# Autodesk Inventor assembly: 101_CompCellScopeAssembly
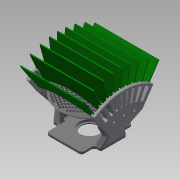
[picture p0: Inventor's stored thumbnail of the model, 180x180]
Saved by Autodesk Inventor 2015 (Build 190159000, 159)
## iProperties
Created: 2015-01-06
Part Number: 101_CompCellScopeAssembly
Document SubType Name: Assembly
Designer: Zack
Author: Zack
## Documents named in this file (6)
- C:\Users\Zack\Dropbox\LED_Array_CellScope\OpenSource\CAD Designs\Inventor\For Submission\101_CompCellScopeAssembly.iam
- C:\Users\Zack\Dropbox\LED_Array_CellScope\OpenSource\CAD Designs\Inventor\For Submission\102_CompCellScopeDome.ipt
- C:\Users\Zack\Dropbox\LED_Array_CellScope\OpenSource\CAD Designs\Inventor\For Submission\103_CompCellScopeStage.ipt
- C:\Users\Zack\Dropbox\LED_Array_CellScope\OpenSource\CAD Designs\Inventor\For Submission\104_CompCellScopeBoardHolder.ipt
- C:\Users\Zack\Dropbox\LED_Array_CellScope\OpenSource\CAD Designs\Inventor\For Submission\901_CompCellScopeBoard_FORPICS.ipt
- C:\Users\Zack\Dropbox\LED_Array_CellScope\OpenSource\CAD Designs\Inventor\For Submission\902_CompCellScopeLED_FORPICS.ipt
## Components (14 placed, 5 different names)
1. 102_CompCellScopeDome:1 — Mate:1, Angle:1, Angle:2, Mate:2, Mate:3, Mate:4, Mate:38, Mate:39
2. 103_CompCellScopeStage:1 — Mate:2, Mate:3, Mate:4, Mate:6
3. 104_CompCellScopeBoardHolder:1 — Mate:6, Mate:7, Angle:3, Mate:27, Mate:28, Mate:29, Mate:30, Mate:31, Mate:32, Mate:34, Mate:35
4. 104_CompCellScopeBoardHolder:2 — Mate:8, Mate:9, Flush:1, Mate:10, Mate:11, Mate:12, Mate:13, Mate:14, Mate:15, Mate:16, Mate:17, Mate:18, Mate:19, Mate:20, Mate:21, Mate:22, Mate:23, Mate:24, Mate:25, Mate:26, Mate:33, Mate:36, Mate:37
5. 901_CompCellScopeBoard_FORPICS:1 — Mate:10, Mate:11, Mate:12
6. 901_CompCellScopeBoard_FORPICS:2 — Mate:17, Mate:18, Mate:19
7. 901_CompCellScopeBoard_FORPICS:3 — Mate:20, Mate:21, Mate:22
8. 901_CompCellScopeBoard_FORPICS:4 — Mate:13, Mate:14, Mate:15, Mate:16
9. 901_CompCellScopeBoard_FORPICS:5 — Mate:23, Mate:24, Mate:25
10. 901_CompCellScopeBoard_FORPICS:6 — Mate:31, Mate:32, Mate:36
11. 901_CompCellScopeBoard_FORPICS:7 — Mate:29, Mate:30, Mate:37
12. 901_CompCellScopeBoard_FORPICS:8 — Mate:26, Mate:27, Mate:28
13. 901_CompCellScopeBoard_FORPICS:9 — Mate:33, Mate:34, Mate:35
14. 902_CompCellScopeLED_FORPICS:1 — Mate:38, Mate:39
## Relationships (42: Mate 38, Angle 3, Flush 1)
- Mate:1: 102_CompCellScopeDome:1
- Angle:1 (0 deg): 102_CompCellScopeDome:1
- Angle:2 (0 deg): 102_CompCellScopeDome:1
- Mate:2: 102_CompCellScopeDome:1 ↔ 103_CompCellScopeStage:1
- Mate:3: 102_CompCellScopeDome:1 ↔ 103_CompCellScopeStage:1
- Mate:4: 102_CompCellScopeDome:1 ↔ 103_CompCellScopeStage:1
- Mate:6: 103_CompCellScopeStage:1 ↔ 104_CompCellScopeBoardHolder:1
- Mate:7: 104_CompCellScopeBoardHolder:1
- Angle:3 (0 deg): 104_CompCellScopeBoardHolder:1
- Mate:8: 104_CompCellScopeBoardHolder:2
- Mate:9: 104_CompCellScopeBoardHolder:2
- Flush:1: 104_CompCellScopeBoardHolder:2
- Mate:10: 104_CompCellScopeBoardHolder:2 ↔ 901_CompCellScopeBoard_FORPICS:1
- Mate:11: 104_CompCellScopeBoardHolder:2 ↔ 901_CompCellScopeBoard_FORPICS:1
- Mate:12: 104_CompCellScopeBoardHolder:2 ↔ 901_CompCellScopeBoard_FORPICS:1
- Mate:13: 104_CompCellScopeBoardHolder:2 ↔ 901_CompCellScopeBoard_FORPICS:4
- Mate:14: 104_CompCellScopeBoardHolder:2 ↔ 901_CompCellScopeBoard_FORPICS:4
- Mate:15: 104_CompCellScopeBoardHolder:2 ↔ 901_CompCellScopeBoard_FORPICS:4
- Mate:16: 104_CompCellScopeBoardHolder:2 ↔ 901_CompCellScopeBoard_FORPICS:4
- Mate:17: 104_CompCellScopeBoardHolder:2 ↔ 901_CompCellScopeBoard_FORPICS:2
- Mate:18: 104_CompCellScopeBoardHolder:2 ↔ 901_CompCellScopeBoard_FORPICS:2
- Mate:19: 104_CompCellScopeBoardHolder:2 ↔ 901_CompCellScopeBoard_FORPICS:2
- Mate:20: 104_CompCellScopeBoardHolder:2 ↔ 901_CompCellScopeBoard_FORPICS:3
- Mate:21: 104_CompCellScopeBoardHolder:2 ↔ 901_CompCellScopeBoard_FORPICS:3
- Mate:22: 104_CompCellScopeBoardHolder:2 ↔ 901_CompCellScopeBoard_FORPICS:3
- Mate:23: 104_CompCellScopeBoardHolder:2 ↔ 901_CompCellScopeBoard_FORPICS:5
- Mate:24: 104_CompCellScopeBoardHolder:2 ↔ 901_CompCellScopeBoard_FORPICS:5
- Mate:25: 104_CompCellScopeBoardHolder:2 ↔ 901_CompCellScopeBoard_FORPICS:5
- Mate:26: 104_CompCellScopeBoardHolder:2 ↔ 901_CompCellScopeBoard_FORPICS:8
- Mate:27: 104_CompCellScopeBoardHolder:1 ↔ 901_CompCellScopeBoard_FORPICS:8
- Mate:28: 104_CompCellScopeBoardHolder:1 ↔ 901_CompCellScopeBoard_FORPICS:8
- Mate:29: 104_CompCellScopeBoardHolder:1 ↔ 901_CompCellScopeBoard_FORPICS:7
- Mate:30: 104_CompCellScopeBoardHolder:1 ↔ 901_CompCellScopeBoard_FORPICS:7
- Mate:31: 104_CompCellScopeBoardHolder:1 ↔ 901_CompCellScopeBoard_FORPICS:6
- Mate:32: 104_CompCellScopeBoardHolder:1 ↔ 901_CompCellScopeBoard_FORPICS:6
- Mate:33: 104_CompCellScopeBoardHolder:2 ↔ 901_CompCellScopeBoard_FORPICS:9
- Mate:34: 104_CompCellScopeBoardHolder:1 ↔ 901_CompCellScopeBoard_FORPICS:9
- Mate:35: 104_CompCellScopeBoardHolder:1 ↔ 901_CompCellScopeBoard_FORPICS:9
- Mate:36: 104_CompCellScopeBoardHolder:2 ↔ 901_CompCellScopeBoard_FORPICS:6
- Mate:37: 104_CompCellScopeBoardHolder:2 ↔ 901_CompCellScopeBoard_FORPICS:7
- Mate:38: 102_CompCellScopeDome:1 ↔ 902_CompCellScopeLED_FORPICS:1
- Mate:39: 102_CompCellScopeDome:1 ↔ 902_CompCellScopeLED_FORPICS:1
